# Autodesk Inventor assembly: endAssembly
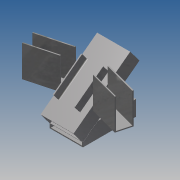
[picture p0: Inventor's stored thumbnail of the model, 180x180]
Saved by Autodesk Inventor 2013 SP2 (Build 170200200, 200)
## iProperties
Created: 2013-12-03
Part Number: endAssembly
Document SubType Name: Assembly
Designer: Dave
Author: Dave
## Documents named in this file (6)
- C:\Users\Dave\Desktop\hera-cad\support\endAssembly.iam
- C:\Users\Dave\Desktop\hera-cad\support\endHoriz.ipt
- C:\Users\Dave\Desktop\hera-cad\support\end37.ipt
- C:\Users\Dave\Desktop\hera-cad\support\endVert1.ipt
- C:\Users\Dave\Desktop\hera-cad\support\endVert2.ipt
- C:\Users\Dave\Desktop\hera-cad\support\end37channel.ipt
## Components (5 placed, 5 different names)
1. endHoriz:1 — Mate:1, Flush:1, Flush:3
2. end37:1 — Mate:1, Mate:5, Mate:6, Mate:7, Flush:3, Flush:4, Flush:5
3. endVert1:1 — Flush:1, Mate:7, Flush:2
4. endVert2:1 — Mate:6, Flush:2
5. end37channel:1 — Mate:5, Flush:4, Flush:5
## Relationships (9: Flush 5, Mate 4)
- Mate:1: endHoriz:1 ↔ end37:1
- Mate:5: end37:1 ↔ end37channel:1
- Flush:1 (-76.2 mm): endHoriz:1 ↔ endVert1:1
- Mate:6: end37:1 ↔ endVert2:1
- Mate:7: end37:1 ↔ endVert1:1
- Flush:2: endVert1:1 ↔ endVert2:1
- Flush:3: endHoriz:1 ↔ end37:1
- Flush:4 (44.45 mm): end37:1 ↔ end37channel:1
- Flush:5 (-16.51 mm): end37:1 ↔ end37channel:1
